# Autodesk Inventor assembly: SoapAssembly
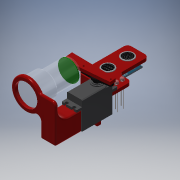
[picture p0: Inventor's stored thumbnail of the model, 180x180]
Saved by Autodesk Inventor 2018.3 (Build 223284000, 284)
## iProperties
Created: 2020-03-24
Part Number: SoapAssembly
Document SubType Name: Assembly
Designer: Ivan
Author: Ivan
## Documents named in this file (11)
- C:\Users\Ivan\Documents\GitHub\Soap-dispenser\3D Model\SoapAssembly.iam
- C:\Users\Ivan\Documents\GitHub\Soap-dispenser\3D Model\ServoSupport.ipt
- C:\Users\Ivan\Documents\GitHub\Soap-dispenser\3D Model\Servo MG995.ipt
- C:\Users\Ivan\Documents\GitHub\Soap-dispenser\3D Model\DispenserHead.ipt
- C:\Users\Ivan\Documents\GitHub\Soap-dispenser\3D Model\ServoArm2.ipt
- C:\Users\Ivan\Documents\GitHub\Soap-dispenser\3D Model\HC-SR04.ipt
- C:\Users\Ivan\Documents\GitHub\Soap-dispenser\3D Model\UltrasonicBase.ipt
- C:\Users\Ivan\Documents\GitHub\Soap-dispenser\3D Model\LED 5mm.ipt
- C:\Users\Ivan\Documents\GitHub\Soap-dispenser\3D Model\Arduino Pro Mini -Detailed -Blue.ipt
- C:\Users\Ivan\Documents\GitHub\Soap-dispenser\3D Model\ArmExtension.ipt
- C:\Users\Ivan\Documents\GitHub\Soap-dispenser\3D Model\MovingPlane.ipt
## Components (11 placed, 10 different names)
1. ServoSupport:1 — Mate:1, Flush:1, Mate:2, Mate:3, Mate:4, Mate:20
2. Servo MG995:1 — Mate:1, Flush:1, Mate:2, Insert:1, Mate:5, Flush:2, Mate:6, Angle:1, Angle:2
3. DispenserHead:1 — Mate:3, Mate:4
4. ServoArm2:1 — Insert:1, Mate:17, Mate:18, Mate:19
5. HC-SR04:1 — Angle:1, Mate:7, Mate:8
6. UltrasonicBase:1 — Mate:5, Flush:2, Mate:6, Mate:7, Mate:8, Mate:9, Mate:10, Mate:11, Mate:12, Mate:14, Mate:15, Mate:16
7. LED 5mm:1 — Mate:9, Mate:11
8. LED 5mm:2 — Mate:10, Mate:12
9. Arduino Pro Mini -Detailed -Blue:1 — Angle:2, Mate:14, Mate:15, Mate:16
10. ArmExtension:1 — Mate:17, Mate:18, Mate:19, Tangent:1
11. MovingPlane:1 — Tangent:1, Mate:20
## Relationships (25: Mate 19, Flush 2, Angle 2, Insert 1, Tangent 1)
- Mate:1: ServoSupport:1 ↔ Servo MG995:1
- Flush:1: ServoSupport:1 ↔ Servo MG995:1
- Mate:2: ServoSupport:1 ↔ Servo MG995:1
- Mate:3: ServoSupport:1 ↔ DispenserHead:1
- Mate:4: ServoSupport:1 ↔ DispenserHead:1
- Insert:1: Servo MG995:1 ↔ ServoArm2:1
- Mate:5: Servo MG995:1 ↔ UltrasonicBase:1
- Flush:2: Servo MG995:1 ↔ UltrasonicBase:1
- Mate:6: Servo MG995:1 ↔ UltrasonicBase:1
- Angle:1 (0 deg): Servo MG995:1 ↔ HC-SR04:1
- Mate:7: HC-SR04:1 ↔ UltrasonicBase:1
- Mate:8: HC-SR04:1 ↔ UltrasonicBase:1
- Mate:9: UltrasonicBase:1 ↔ LED 5mm:1
- Mate:10: UltrasonicBase:1 ↔ LED 5mm:2
- Mate:11: UltrasonicBase:1 ↔ LED 5mm:1
- Mate:12: UltrasonicBase:1 ↔ LED 5mm:2
- Angle:2 (180 deg): Servo MG995:1 ↔ Arduino Pro Mini -Detailed -Blue:1
- Mate:14: UltrasonicBase:1 ↔ Arduino Pro Mini -Detailed -Blue:1
- Mate:15: UltrasonicBase:1 ↔ Arduino Pro Mini -Detailed -Blue:1
- Mate:16: UltrasonicBase:1 ↔ Arduino Pro Mini -Detailed -Blue:1
- Mate:17: ServoArm2:1 ↔ ArmExtension:1
- Mate:18: ServoArm2:1 ↔ ArmExtension:1
- Mate:19: ServoArm2:1 ↔ ArmExtension:1
- Tangent:1: ArmExtension:1 ↔ MovingPlane:1
- Mate:20: ServoSupport:1 ↔ MovingPlane:1
